# Autodesk Inventor assembly: GearToScrew
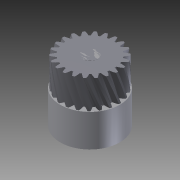
[picture p0: Inventor's stored thumbnail of the model, 180x180]
Saved by Autodesk Inventor 2012 (Build 160160000, 160)
## iProperties
Created: 2011-10-20
Part Number: GearToScrew
Document SubType Name: Assembly
Designer: KuttaA
Author: KuttaA
## Documents named in this file (3)
- C:\Users\KuttaA\Dropbox\Hexapod Research\Leg Design\Other Parts\GearToScrew.iam
- C:\Users\KuttaA\Dropbox\Hexapod Research\Leg Design\Other Parts\GearToScrew.ipt
- C:\Users\KuttaA\Dropbox\Hexapod Research\Leg Design\Other Parts\NewScrewDrive\Design Accelerator\Spur Gear12.ipt
## Components (2 placed, 2 different names)
1. GearToScrew:1 — Mate:1, Mate:2
2. Spur Gear1:1 — Mate:1, Mate:2
## Relationships (2: Mate 2)
- Mate:1: GearToScrew:1 ↔ Spur Gear1:1
- Mate:2: GearToScrew:1 ↔ Spur Gear1:1
